# Autodesk Inventor assembly: main_frame_assem
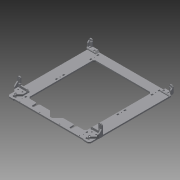
[picture p0: Inventor's stored thumbnail of the model, 180x180]
Saved by Autodesk Inventor 2015 (Build 190159000, 159)
## iProperties
Created: 2015-06-01
Part Number: main_frame_assem
Document SubType Name: Assembly
Designer: X
Author: X
## Documents named in this file (16)
- C:\Users\marc\Documents\GitHub\Prusa_i3\main_frame_assem.iam
- C:\Users\marc\Documents\GitHub\Prusa_i3\frame\main_frame.ipt
- C:\Users\marc\Documents\GitHub\Prusa_i3\3d_printer_part\z-axis-top.ipt
- C:\Users\marc\Documents\GitHub\Prusa_i3\3d_printer_part\z-axis-bottom.ipt
- C:\Users\marc\Documents\GitHub\Prusa_i3\3d_printer_part\z-axis-top_MIR.ipt
- C:\Users\marc\Documents\GitHub\Prusa_i3\3d_printer_part\z-axis-bottom_MIR.ipt
- C:\Users\marc\Documents\GitHub\Prusa_i3\main_frame_assem\Design Accelerator\Bolted Connection1.iam
- C:\Users\marc\Documents\GitHub\Prusa_i3\main_frame_assem\Design Accelerator\Bolted Connection2.iam
- C:\Users\marc\Documents\GitHub\Prusa_i3\main_frame_assem\Design Accelerator\Bolted Connection3.iam
- C:\Users\marc\Documents\GitHub\Prusa_i3\main_frame_assem\Design Accelerator\Bolted Connection4.iam
- C:\Users\marc\Documents\GitHub\Prusa_i3\main_frame_assem\Design Accelerator\Bolted Connection5.iam
- C:\Users\marc\Documents\GitHub\Prusa_i3\main_frame_assem\Design Accelerator\Bolted Connection6.iam
- C:\Users\marc\Documents\GitHub\Prusa_i3\main_frame_assem\Design Accelerator\Bolted Connection7.iam
- C:\Users\marc\Documents\GitHub\Prusa_i3\main_frame_assem\Design Accelerator\Bolted Connection8.iam
- C:\Users\marc\Documents\GitHub\Prusa_i3\main_frame_assem\Design Accelerator\Bolted Connection9.iam
- C:\Users\marc\Documents\GitHub\Prusa_i3\main_frame_assem\Design Accelerator\Bolted Connection10.iam
## Components (15 placed, 6 different names)
1. main_frame:1 — Mate:1, Cylindrical:1, Cylindrical:2, Mate:2, Cylindrical:3, Cylindrical:4, Mate:3, Mate:4, Flush:2, Mate:5, Mate:6, Cylindrical:5, Insert:1, Mate:7, Mate:8, Insert:2, Cylindrical:6, Mate:16, Mate:18, Mate:20, Mate:22, Mate:24, Mate:26, Mate:28
2. z-axis-top:1 — Mate:1, Cylindrical:1, Cylindrical:2, Mate:25, Mate:27
3. z-axis-bottom:1 — Mate:2, Cylindrical:3, Cylindrical:4, Mate:9, Mate:10, Mate:11, Mate:12, Mate:13, Mate:14
4. z-axis-top_MIR:1 — Mate:8, Insert:2, Cylindrical:6, Mate:21, Mate:23
5. z-axis-bottom_MIR:1 — Cylindrical:5, Insert:1, Mate:7, Mate:15, Mate:17, Mate:19
6. Bolted Connection:1 [sub-assembly] — Mate:9, Mate:10
7. Bolted Connection:2 [sub-assembly] — Mate:11, Mate:12
8. Bolted Connection:3 [sub-assembly] — Mate:13, Mate:14
9. Bolted Connection:4 [sub-assembly] — Mate:15, Mate:16
10. Bolted Connection:5 [sub-assembly] — Mate:17, Mate:18
11. Bolted Connection:6 [sub-assembly] — Mate:19, Mate:20
12. Bolted Connection:7 [sub-assembly] — Mate:21, Mate:22
13. Bolted Connection:8 [sub-assembly] — Mate:23, Mate:24
14. Bolted Connection:9 [sub-assembly] — Mate:25, Mate:26
15. Bolted Connection:10 [sub-assembly] — Mate:27, Mate:28
## Relationships (38: Mate 28, CylindricalJoint 6, Flush 2, Insert 2)
- Mate:1: main_frame:1 ↔ z-axis-top:1
- Cylindrical:1: main_frame:1 ↔ z-axis-top:1
- Cylindrical:2: main_frame:1 ↔ z-axis-top:1
- Mate:2: main_frame:1 ↔ z-axis-bottom:1
- Cylindrical:3: main_frame:1 ↔ z-axis-bottom:1
- Cylindrical:4: main_frame:1 ↔ z-axis-bottom:1
- Mate:3: main_frame:1
- Mate:4: main_frame:1
- Flush:1 (185 mm)
- Flush:2: main_frame:1
- Mate:5: main_frame:1
- Mate:6: main_frame:1
- Cylindrical:5: main_frame:1 ↔ z-axis-bottom_MIR:1
- Insert:1: main_frame:1 ↔ z-axis-bottom_MIR:1
- Mate:7: main_frame:1 ↔ z-axis-bottom_MIR:1
- Mate:8: main_frame:1 ↔ z-axis-top_MIR:1
- Insert:2: main_frame:1 ↔ z-axis-top_MIR:1
- Cylindrical:6: main_frame:1 ↔ z-axis-top_MIR:1
- Mate:9: z-axis-bottom:1 ↔ Bolted Connection:1
- Mate:10: z-axis-bottom:1 ↔ Bolted Connection:1
- Mate:11: z-axis-bottom:1 ↔ Bolted Connection:2
- Mate:12: z-axis-bottom:1 ↔ Bolted Connection:2
- Mate:13: z-axis-bottom:1 ↔ Bolted Connection:3
- Mate:14: z-axis-bottom:1 ↔ Bolted Connection:3
- Mate:15: z-axis-bottom_MIR:1 ↔ Bolted Connection:4
- Mate:16: main_frame:1 ↔ Bolted Connection:4
- Mate:17: z-axis-bottom_MIR:1 ↔ Bolted Connection:5
- Mate:18: main_frame:1 ↔ Bolted Connection:5
- Mate:19: z-axis-bottom_MIR:1 ↔ Bolted Connection:6
- Mate:20: main_frame:1 ↔ Bolted Connection:6
- Mate:21: z-axis-top_MIR:1 ↔ Bolted Connection:7
- Mate:22: main_frame:1 ↔ Bolted Connection:7
- Mate:23: z-axis-top_MIR:1 ↔ Bolted Connection:8
- Mate:24: main_frame:1 ↔ Bolted Connection:8
- Mate:25: z-axis-top:1 ↔ Bolted Connection:9
- Mate:26: main_frame:1 ↔ Bolted Connection:9
- Mate:27: z-axis-top:1 ↔ Bolted Connection:10
- Mate:28: main_frame:1 ↔ Bolted Connection:10
